# Autodesk Inventor assembly: Module Assembly
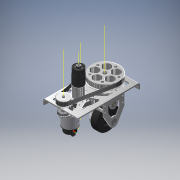
[picture p0: Inventor's stored thumbnail of the model, 180x180]
Saved by Autodesk Inventor 2019.4 (Build 234330000, 330)
## iProperties
Created: 2019-11-29
Part Number: Module Assembly
Document SubType Name: Assembly
Designer: admin
Mass: 4028.68 g
Surface Area: 4867.45 cm^2
Volume: 1353.44 cm^3
Density: 2.97662 g/cm^3
Author: admin
## Documents named in this file (25)
- C:\Users\admin\Desktop\FRC 2020 Engineering\Swerve Module\Module Assembly.iam
- C:\Users\admin\Desktop\FRC 2020 Engineering\Swerve Module\100mm Traction Wheel StandIn.ipt
- C:\Users\admin\Desktop\FRC 2020 Engineering\Swerve Module\Falcon_500_Powered_by_Talon_FX_217-6515.iam
- C:\Users\admin\Desktop\FRC 2020 Engineering\Swerve Module\U Bend.ipt
- C:\Users\admin\Desktop\FRC 2020 Engineering\Swerve Module\Bearing.ipt
- C:\Users\admin\Desktop\FRC 2020 Engineering\Swerve Module\Module Assembly\Design Accelerator\Synchronous Belts Transmission3.iam
- C:\Users\admin\Desktop\FRC 2020 Engineering\Swerve Module\Module Assembly\Design Accelerator\Synchronous Belts Transmission4.iam
- C:\Users\admin\Desktop\FRC 2020 Engineering\Swerve Module\Top Plate.ipt
- C:\Users\admin\Desktop\FRC 2020 Engineering\Swerve Module\F6802.ipt
- C:\Users\admin\Desktop\FRC 2020 Engineering\Swerve Module\Main Vert Axle.ipt
- C:\Users\admin\Desktop\FRC 2020 Engineering\Swerve Module\Module Assembly\Design Accelerator\Bevel Gears2.iam
- C:\Users\admin\Desktop\FRC 2020 Engineering\Swerve Module\Module Assembly\Design Accelerator\Spur Gears4.iam
- C:\Users\admin\Desktop\FRC 2020 Engineering\Swerve Module\30t_Aluminum_Spur_Gear_20_DP_1_2_Hex_Bore_217-2705.ipt
- C:\Users\admin\Desktop\FRC 2020 Engineering\Swerve Module\14T_Steel_Spur_Gear_20_DP_Falcon_Motor_217-6922.ipt
- C:\Users\admin\Desktop\FRC 2020 Engineering\Swerve Module\EB38S6 Encoder.ipt
- C:\Users\admin\Desktop\FRC 2020 Engineering\Swerve Module\F6800Z 10mm ID Flange.ipt
- C:\Users\admin\Desktop\FRC 2020 Engineering\Swerve Module\Bevel - Spur Axle.ipt
- C:\Users\admin\Desktop\FRC 2020 Engineering\Swerve Module\Wheel - Spur Axle.ipt
- C:\Users\admin\Desktop\FRC 2020 Engineering\Swerve Module\27-1 Gearbox.ipt
- C:\Users\admin\Desktop\FRC 2020 Engineering\Swerve Module\775pro_217-4347.ipt
- C:\Users\admin\Desktop\FRC 2020 Engineering\Swerve Module\Gear - Drive Axle.ipt
- C:\Users\admin\Desktop\FRC 2020 Engineering\GitHub\7738-CAD-prep\775 Mounting plate.ipt
- C:\Users\admin\Desktop\FRC 2020 Engineering\Swerve Module\Motor Mount Plate.ipt
- C:\Users\admin\Desktop\FRC 2020 Engineering\Swerve Module\Spacer.ipt
- C:\Users\admin\Desktop\FRC 2020 Engineering\Swerve Module\Spacer 2.ipt
## Components (36 placed, 23 different names)
1. 100mm Traction Wheel StandIn:1
2. Falcon_500_Powered_by_Talon_FX_217-6515:1 [sub-assembly] — Mate:12, Mate:13, Mate:21, Mate:33, Flush:3, Mate:34, Mate:35
3. U Bend:1 — Mate:45, Mate:46, Mate:47, Mate:48, Mate:49, Mate:50, Mate:51, Mate:52
4. Synchronous Belts Transmission:1 [sub-assembly] — Mate:1, Mate:6, Mate:19, Mate:20, Mate:25, Mate:28, Mate:29
5. Synchronous Belts Transmission:2 [sub-assembly] — Mate:14, Mate:22
6. F6802:2
7. F6802:3
8. F6802:4 — Mate:4, Mate:5
9. Main Vert Axle:1 — Mate:3, Mate:4, Mate:5, Flush:1
10. Bevel Gears:2 [sub-assembly] — Mate:2, Mate:3, Flush:1
11. Spur Gears:3 [sub-assembly]
12. 30t_Aluminum_Spur_Gear_20_DP_1_2_Hex_Bore_217-2705:1 — Mate:11, Mate:13, Flush:2, Mate:18
13. 14T_Steel_Spur_Gear_20_DP_Falcon_Motor_217-6922:1 — Mate:12, Flush:2
14. F6800Z 10mm ID Flange:1
15. F6800Z 10mm ID Flange:2
16. Bevel - Spur Axle:2
17. F6802:5
18. Wheel - Spur Axle:1
19. 27-1 Gearbox:1 — Mate:8, Mate:9, Mate:28, Mate:29, Mate:30, Mate:31
20. 775pro_217-4347:1 — Mate:8, Mate:9
21. EB38S6 Encoder:2 — Mate:6, Flush:3
22. F6802:6 — Mate:16
23. F6800Z 10mm ID Flange:3 — Mate:15, Mate:17, Mate:18, Mate:33
24. Gear - Drive Axle:1 — Mate:11, Mate:14, Mate:15, Mate:16, Mate:17, Mate:22
25. Bearing:1 — Mate:1, Mate:2, Mate:19, Mate:20, Mate:24
26. Top Plate:2 — Mate:24, Mate:25
27. 775 Mounting plate:1 — Mate:30, Mate:31
28. Motor Mount Plate:1 — Mate:34, Mate:35, Mate:37, Mate:38, Mate:39, Mate:40
29. Spacer:1 — Mate:37
30. Spacer:2 — Mate:38
31. Spacer:3 — Mate:40
32. Spacer:5 — Mate:39
33. Spacer 2:1 — Mate:47, Mate:49
34. Spacer 2:2 — Mate:48, Mate:50
35. Spacer 2:3 — Mate:46, Mate:52
36. Spacer 2:4 — Mate:45, Mate:51
## Relationships (44: Mate 41, Flush 3)
- Mate:1 (1 mm): Synchronous Belts Transmission:1 ↔ Bearing:1
- Mate:2: Bevel Gears:2 ↔ Bearing:1
- Mate:3: Main Vert Axle:1 ↔ Bevel Gears:2
- Mate:4 (0.2 mm): F6802:4 ↔ Main Vert Axle:1
- Mate:5: F6802:4 ↔ Main Vert Axle:1
- Flush:1 (-0.1 mm): Main Vert Axle:1 ↔ Bevel Gears:2
- Mate:6: Synchronous Belts Transmission:1 ↔ EB38S6 Encoder:2
- Mate:8: 27-1 Gearbox:1 ↔ 775pro_217-4347:1
- Mate:9: 27-1 Gearbox:1 ↔ 775pro_217-4347:1
- Mate:11: 30t_Aluminum_Spur_Gear_20_DP_1_2_Hex_Bore_217-2705:1 ↔ Gear - Drive Axle:1
- Mate:12: Falcon_500_Powered_by_Talon_FX_217-6515:1 ↔ 14T_Steel_Spur_Gear_20_DP_Falcon_Motor_217-6922:1
- Mate:13 (27.94 mm): Falcon_500_Powered_by_Talon_FX_217-6515:1 ↔ 30t_Aluminum_Spur_Gear_20_DP_1_2_Hex_Bore_217-2705:1
- Flush:2 (1 mm): 30t_Aluminum_Spur_Gear_20_DP_1_2_Hex_Bore_217-2705:1 ↔ 14T_Steel_Spur_Gear_20_DP_Falcon_Motor_217-6922:1
- Mate:14: Synchronous Belts Transmission:2 ↔ Gear - Drive Axle:1
- Mate:15: F6800Z 10mm ID Flange:3 ↔ Gear - Drive Axle:1
- Mate:16: F6802:6 ↔ Gear - Drive Axle:1
- Mate:17 (0.2 mm): F6800Z 10mm ID Flange:3 ↔ Gear - Drive Axle:1
- Mate:18 (0.2 mm): 30t_Aluminum_Spur_Gear_20_DP_1_2_Hex_Bore_217-2705:1 ↔ F6800Z 10mm ID Flange:3
- Mate:19: Synchronous Belts Transmission:1 ↔ Bearing:1
- Mate:20: Synchronous Belts Transmission:1 ↔ Bearing:1
- Mate:21: Falcon_500_Powered_by_Talon_FX_217-6515:1
- Mate:22 (0.2 mm): Synchronous Belts Transmission:2 ↔ Gear - Drive Axle:1
- Mate:24 (1 mm): Bearing:1 ↔ Top Plate:2
- Mate:25: Synchronous Belts Transmission:1 ↔ Top Plate:2
- Mate:28: Synchronous Belts Transmission:1 ↔ 27-1 Gearbox:1
- Mate:29 (5.5 mm): Synchronous Belts Transmission:1 ↔ 27-1 Gearbox:1
- Mate:30: 27-1 Gearbox:1 ↔ 775 Mounting plate:1
- Mate:31: 27-1 Gearbox:1 ↔ 775 Mounting plate:1
- Mate:33 (5.2 mm): Falcon_500_Powered_by_Talon_FX_217-6515:1 ↔ F6800Z 10mm ID Flange:3
- Flush:3 (1 mm): Falcon_500_Powered_by_Talon_FX_217-6515:1 ↔ EB38S6 Encoder:2
- Mate:34: Falcon_500_Powered_by_Talon_FX_217-6515:1 ↔ Motor Mount Plate:1
- Mate:35: Falcon_500_Powered_by_Talon_FX_217-6515:1 ↔ Motor Mount Plate:1
- Mate:37: Motor Mount Plate:1 ↔ Spacer:1
- Mate:38: Motor Mount Plate:1 ↔ Spacer:2
- Mate:39: Motor Mount Plate:1 ↔ Spacer:5
- Mate:40: Motor Mount Plate:1 ↔ Spacer:3
- Mate:45: U Bend:1 ↔ Spacer 2:4
- Mate:46: U Bend:1 ↔ Spacer 2:3
- Mate:47: U Bend:1 ↔ Spacer 2:1
- Mate:48: U Bend:1 ↔ Spacer 2:2
- Mate:49 (0.2 mm): U Bend:1 ↔ Spacer 2:1
- Mate:50 (0.2 mm): U Bend:1 ↔ Spacer 2:2
- Mate:51 (0.2 mm): U Bend:1 ↔ Spacer 2:4
- Mate:52 (0.2 mm): U Bend:1 ↔ Spacer 2:3
